# Autodesk Inventor assembly: shuttle cock assembly 2
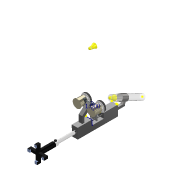
[picture p0: Inventor's stored thumbnail of the model, 180x180]
Saved by Autodesk Inventor 2021 (Build 250183000, 183)
## iProperties
Created: 2021-07-01
Part Number: shuttle cock assembly 2
Document SubType Name: Assembly
Designer: user
Author: user
## Documents named in this file (11)
- C:\Users\user\Desktop\New folder\A.Final Assembly.0013.iam
- C:\Users\user\Desktop\New folder\8.Main Machine Support.ipt
- C:\Users\user\Desktop\New folder\1.DC Motor.ipt
- C:\Users\user\Desktop\New folder\4.Clamps.ipt
- C:\Users\user\Desktop\New folder\6.Shuttle Cock Storage.ipt
- C:\Users\user\Desktop\New folder\7.Shuttle Cock Storage Holder.ipt
- C:\Users\user\Desktop\New folder\9.Stand.ipt
- C:\Users\user\Desktop\New folder\2.DC Motor Holder.ipt
- C:\Users\user\Desktop\New folder\3.DC Motor Wheel.ipt
- C:\Users\user\Desktop\New folder\5.Clamp Base.ipt
- C:\Users\user\Desktop\New folder\10.Shuttle Cock.ipt
## Components (14 placed, 10 different names)
1. 8.Main Machine Support:1 — Mate:1, Mate:2, Mate:3, Mate:6, Mate:7, Mate:8, Mate:13, Mate:14, Mate:16, Mate:17
2. 1.DC Motor:1 — Mate:9, Flush:3, Mate:12, Flush:6, Rotational:1
3. 1.DC Motor:2 — Mate:10, Flush:4, Mate:11, Flush:5
4. 4.Clamps:1 — Mate:5, Flush:2
5. 4.Clamps:2 — Mate:4, Flush:1
6. 6.Shuttle Cock Storage:1 — Mate:15, Mate:18
7. 7.Shuttle Cock Storage Holder:1 — Mate:13, Mate:14, Mate:15
8. 9.Stand:1 — Mate:1, Mate:2
9. 2.DC Motor Holder:1 — Mate:6, Mate:7, Mate:8, Mate:9, Flush:3, Mate:10, Flush:4
10. 3.DC Motor Wheel:1 — Mate:11, Flush:5
11. 3.DC Motor Wheel:2 — Mate:12, Flush:6, Rotational:1, Mate:19
12. 5.Clamp Base:1 — Mate:3, Mate:4, Flush:1, Mate:5, Flush:2, Mate:16, Mate:17
13. 10.Shuttle Cock:1 — Mate:18
14. 10.Shuttle Cock:2 — Mate:19
## Relationships (26: Mate 19, Flush 6, RevoluteJoint 1)
- Mate:1: 8.Main Machine Support:1 ↔ 9.Stand:1
- Mate:2: 8.Main Machine Support:1 ↔ 9.Stand:1
- Mate:3: 8.Main Machine Support:1 ↔ 5.Clamp Base:1
- Mate:4: 4.Clamps:2 ↔ 5.Clamp Base:1
- Flush:1: 4.Clamps:2 ↔ 5.Clamp Base:1
- Mate:5: 4.Clamps:1 ↔ 5.Clamp Base:1
- Flush:2: 4.Clamps:1 ↔ 5.Clamp Base:1
- Mate:6: 8.Main Machine Support:1 ↔ 2.DC Motor Holder:1
- Mate:7: 8.Main Machine Support:1 ↔ 2.DC Motor Holder:1
- Mate:8 (53.34 mm): 8.Main Machine Support:1 ↔ 2.DC Motor Holder:1
- Mate:9: 1.DC Motor:1 ↔ 2.DC Motor Holder:1
- Flush:3 (-19.05 mm): 1.DC Motor:1 ↔ 2.DC Motor Holder:1
- Mate:10: 1.DC Motor:2 ↔ 2.DC Motor Holder:1
- Flush:4 (-19.05 mm): 1.DC Motor:2 ↔ 2.DC Motor Holder:1
- Mate:11: 1.DC Motor:2 ↔ 3.DC Motor Wheel:1
- Flush:5 (-6.35 mm): 1.DC Motor:2 ↔ 3.DC Motor Wheel:1
- Mate:12: 1.DC Motor:1 ↔ 3.DC Motor Wheel:2
- Flush:6 (-6.35 mm): 1.DC Motor:1 ↔ 3.DC Motor Wheel:2
- Mate:13: 8.Main Machine Support:1 ↔ 7.Shuttle Cock Storage Holder:1
- Mate:14: 8.Main Machine Support:1 ↔ 7.Shuttle Cock Storage Holder:1
- Mate:15: 6.Shuttle Cock Storage:1 ↔ 7.Shuttle Cock Storage Holder:1
- Rotational:1 [RevoluteJoint] (-6.35 mm): 1.DC Motor:1 ↔ 3.DC Motor Wheel:2
- Mate:16: 8.Main Machine Support:1 ↔ 5.Clamp Base:1
- Mate:17: 8.Main Machine Support:1 ↔ 5.Clamp Base:1
- Mate:18: 6.Shuttle Cock Storage:1 ↔ 10.Shuttle Cock:1
- Mate:19 (107.95 mm): 3.DC Motor Wheel:2 ↔ 10.Shuttle Cock:2
